# Autodesk Inventor assembly: XM540_NO_BACK
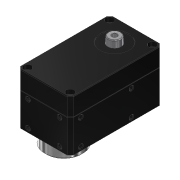
[picture p0: Inventor's stored thumbnail of the model, 180x180]
Saved by Autodesk Inventor 2019.4 (Build 234330000, 330)
## iProperties
Created: 2019-10-19
Part Number: XM540_NO_BACK
Material: 一般
Document SubType Name: Assembly
Designer: y6tada
Author: y6tada
## Documents named in this file (3)
- C:\GrabCAD\Yunit 8\Libs\DYNAMIXEL\XM540\XM540_NO_BACK.iam
- C:\GrabCAD\Yunit 8\Libs\DYNAMIXEL\XM540\XM540_HOUSING_TOP.ipt
- C:\GrabCAD\Yunit 8\Libs\DYNAMIXEL\XM540\XM540_HOUSING_MIDDLE.ipt
## Components (2 placed, 2 different names)
1. XM540_HOUSING_TOP:1 — メイト:1, メイト:2, メイト:3
2. XM540_HOUSING_MIDDLE:1 — メイト:1, メイト:2, メイト:3
## Relationships (3: Mate 3)
- メイト:1 [Mate]: XM540_HOUSING_TOP:1 ↔ XM540_HOUSING_MIDDLE:1
- メイト:2 [Mate]: XM540_HOUSING_TOP:1 ↔ XM540_HOUSING_MIDDLE:1
- メイト:3 [Mate]: XM540_HOUSING_TOP:1 ↔ XM540_HOUSING_MIDDLE:1
